# Autodesk Inventor assembly: цепь_MIR_MIR1
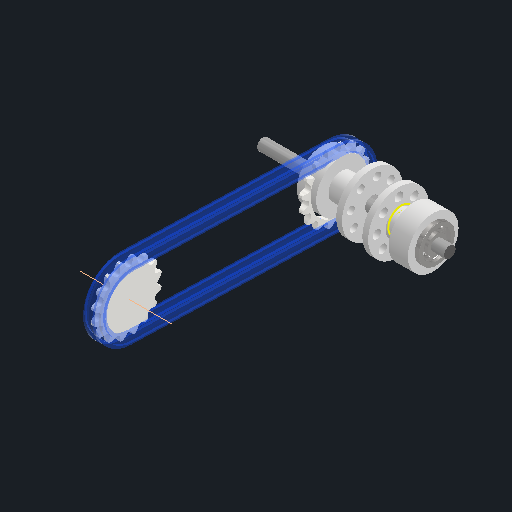
[picture p0: Inventor's stored thumbnail of the model, 512x512]
Saved by Autodesk Inventor 2025 (Build 290162000, 162)
## iProperties
Created: 2024-07-09
Part Number: цепь_MIR_MIR1
Document SubType Name: Assembly
Designer: GameHD
Author: Phantom
## Documents named in this file (6)
- C:\Users\GameHD\Desktop\что-то нужное\Phantom16950\цепь_MIR_MIR1.iam
- C:\Users\GameHD\Desktop\что-то нужное\Phantom16950\Цепной привод2_MIR_MIR.iam
- C:\Users\GameHD\Desktop\что-то нужное\Phantom16950\втулка для подш 2 часть_MIR_MIR.ipt
- C:\Users\GameHD\Desktop\что-то нужное\Phantom16950\втулка для подш_MIR_MIR1.ipt
- C:\Users\GameHD\Desktop\что-то нужное\Phantom16950\Деталь_64_MIR_MIR.ipt
- C:\Users\GameHD\Desktop\что-то нужное\Phantom16950\BS 290 SKF - SKF 626-RZ_MIR_MIR.ipt
## Components (6 placed, 5 different names)
1. Цепной привод2_MIR_MIR:1 [sub-assembly]
2. втулка для подш 2 часть_MIR_MIR:1 — Совмещение:12, Совмещение:11, Заподлицо:2, Совмещение:15
3. втулка для подш_MIR_MIR1:1 — Совмещение:12
4. Деталь_64_MIR_MIR:1 — Совмещение:11, Заподлицо:2, Совмещение:14, Совмещение:10
5. BS 290 SKF - SKF 626-RZ_MIR_MIR:1 — Совмещение:14, Совмещение:15
6. BS 290 SKF - SKF 626-RZ_MIR_MIR:2 — Совмещение:10
## Relationships (6: Mate 5, Flush 1)
- Совмещение:12 [Mate]: втулка для подш 2 часть_MIR_MIR:1 ↔ втулка для подш_MIR_MIR1:1
- Совмещение:11 [Mate]: втулка для подш 2 часть_MIR_MIR:1 ↔ Деталь_64_MIR_MIR:1
- Заподлицо:2 [Flush] (10.245 mm): втулка для подш 2 часть_MIR_MIR:1 ↔ Деталь_64_MIR_MIR:1
- Совмещение:14 [Mate]: Деталь_64_MIR_MIR:1 ↔ BS 290 SKF - SKF 626-RZ_MIR_MIR:1
- Совмещение:15 [Mate]: втулка для подш 2 часть_MIR_MIR:1 ↔ BS 290 SKF - SKF 626-RZ_MIR_MIR:1
- Совмещение:10 [Mate]: Деталь_64_MIR_MIR:1 ↔ BS 290 SKF - SKF 626-RZ_MIR_MIR:2
